# Autodesk Inventor assembly: boxing_MIR
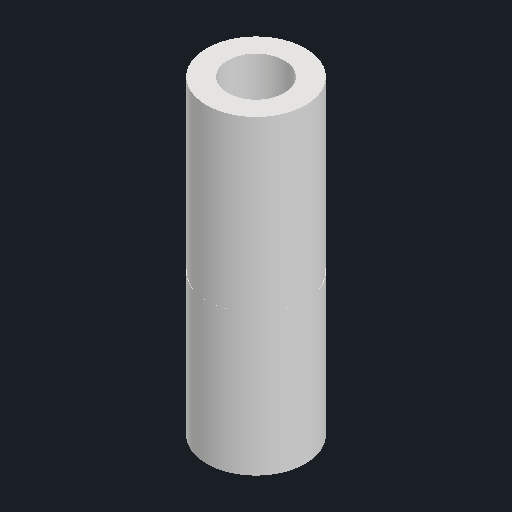
[picture p0: Inventor's stored thumbnail of the model, 512x512]
Saved by Autodesk Inventor 2024 (Build 280153000, 153)
## iProperties
Created: 2024-01-04
Part Number: boxing_MIR
Document SubType Name: Assembly
Designer: macbook
Author: macbook
## Documents named in this file (3)
- \\Mac\Home\Desktop\code\1599V-VRC\Cad\Assembly\boxing_MIR.iam
- \\Mac\Home\Desktop\code\1599V-VRC\Cad\Assembly\10mm spacer_MIR.ipt
- \\Mac\Home\Desktop\code\1599V-VRC\Cad\Assembly\12mm spacer_MIR.ipt
## Components (2 placed, 2 different names)
1. 10mm spacer_MIR:1 — Insert:1
2. 12mm spacer_MIR:1 — Insert:1
## Relationships (1: Insert 1)
- Insert:1: 10mm spacer_MIR:1 ↔ 12mm spacer_MIR:1
